# Autodesk Inventor assembly: ensemble 1
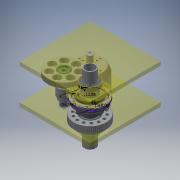
[picture p0: Inventor's stored thumbnail of the model, 180x180]
Saved by Autodesk Inventor 2018.1 (Build 221171000, 171)
## iProperties
Created: 2022-06-30
Part Number: ensemble 1
Document SubType Name: Assembly
Designer: Bureau
Author: Bureau
## Documents named in this file (6)
- C:\Users\Bureau\Mon Drive\Manu\USINAGE\MoteurVelo\ensemble 1.iam
- C:\Users\Bureau\Mon Drive\Manu\USINAGE\MoteurVelo\cote droit.ipt
- C:\Users\Bureau\Mon Drive\Manu\USINAGE\MoteurVelo\Arbre primaire\Assembly1.iam
- C:\Users\Bureau\Mon Drive\Manu\USINAGE\MoteurVelo\Arbre secondaire\Assembly3.iam
- C:\Users\Bureau\Mon Drive\Manu\USINAGE\MoteurVelo\cote gauche.ipt
- C:\Users\Bureau\Mon Drive\Manu\USINAGE\MoteurVelo\Moteur\moteur.iam
## Components (5 placed, 5 different names)
1. cote droit:1 — Mate:1, Mate:2, Mate:3, Mate:4, Flush:1, Mate:8
2. Assembly1:1 [sub-assembly] — Mate:1, Mate:2, Mate:5, Mate:6
3. Assembly3:1 [sub-assembly] — Mate:3, Mate:4
4. cote gauche:1 — Mate:5, Flush:1, Mate:6, Mate:7
5. moteur:1 [sub-assembly] — Mate:7, Mate:8
## Relationships (9: Mate 8, Flush 1)
- Mate:1: cote droit:1 ↔ Assembly1:1
- Mate:2: cote droit:1 ↔ Assembly1:1
- Mate:3: cote droit:1 ↔ Assembly3:1
- Mate:4 (2 mm): cote droit:1 ↔ Assembly3:1
- Mate:5: Assembly1:1 ↔ cote gauche:1
- Flush:1: cote droit:1 ↔ cote gauche:1
- Mate:6: Assembly1:1 ↔ cote gauche:1
- Mate:7: cote gauche:1 ↔ moteur:1
- Mate:8 (2 mm): cote droit:1 ↔ moteur:1
